# Autodesk Inventor assembly: Assemblyclaw pulley thing
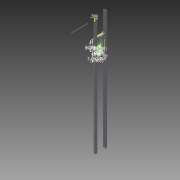
[picture p0: Inventor's stored thumbnail of the model, 180x180]
Saved by Autodesk Inventor 2015 (Build 190159000, 159)
## iProperties
Created: 2015-01-14
Part Number: Assemblyclaw pulley thing
Document SubType Name: Assembly
Designer: mastkee16
Author: mastkee16
## Documents named in this file (8)
- \\lhssvr02\Homedirs\Robotics Club\Hardware\CAD\claw\Assemblyclaw pulley thing.iam
- \\lhssvr02\Homedirs\Robotics Club\Hardware\CAD\claw\trolley plate.ipt
- \\lhssvr02\Homedirs\Robotics Club\Hardware\CAD\claw\wheel.ipt
- \\lhssvr02\Homedirs\Robotics Club\Hardware\CAD\claw\.313 peg.ipt
- \\lhssvr02\Homedirs\Robotics Club\Hardware\CAD\claw\c hannel.ipt
- \\lhssvr02\Homedirs\Robotics Club\Hardware\CAD\claw\motor.ipt
- \\lhssvr02\Homedirs\Robotics Club\Hardware\CAD\claw\#6 screw.ipt
- \\lhssvr02\Homedirs\Robotics Club\Hardware\CAD\claw\Hexagon Rod.ipt
## Components (17 placed, 7 different names)
1. trolley plate:1
2. wheel:1
3. wheel:2
4. wheel:3
5. wheel:4
6. .313 peg:1
7. .313 peg:2
8. .313 peg:3
9. .313 peg:4
10. c hannel:1 — Mate:5, Flush:1, Mate:6
11. c hannel:2 — Mate:6
12. motor:1
13. #6 screw:1
14. #6 screw:2
15. #6 screw:3
16. #6 screw:4
17. Hexagon Rod:1
## Relationships (24: Insert 12, Mate 6, Tangent 5, Flush 1)
- [Insert] (-38.1 mm): trolley plate:1 ↔ .313 peg:1
- [Insert] (-38.1 mm): trolley plate:1 ↔ .313 peg:2
- [Insert] (-38.1 mm): trolley plate:1 ↔ .313 peg:3
- [Insert] (-38.1 mm): trolley plate:1 ↔ .313 peg:4
- [Insert] (-7.747 mm): wheel:2 ↔ .313 peg:1
- [Insert] (-7.747 mm): wheel:1 ↔ .313 peg:2
- [Insert] (7.747 mm): wheel:4 ↔ .313 peg:4
- [Insert] (7.747 mm): wheel:3 ↔ .313 peg:3
- [Mate]: wheel:1 ↔ c hannel:2
- [Mate]: wheel:4 ↔ c hannel:2
- [Tangent]: wheel:4 ↔ c hannel:2
- [Tangent]: wheel:1 ↔ c hannel:2
- [Tangent]: wheel:2 ↔ c hannel:1
- [Tangent]: wheel:3 ↔ c hannel:1
- [Mate]: wheel:3 ↔ c hannel:1
- [Insert]: trolley plate:1 ↔ #6 screw:2
- [Insert]: trolley plate:1 ↔ #6 screw:4
- [Insert]: trolley plate:1 ↔ #6 screw:3
- [Insert]: trolley plate:1 ↔ #6 screw:1
- [Tangent]: trolley plate:1 ↔ motor:1
- [Mate]: trolley plate:1 ↔ motor:1
- Mate:5: c hannel:1
- Flush:1: c hannel:1
- Mate:6: c hannel:1 ↔ c hannel:2
## Named parameters: d15_d20 = 0 mm
